# Autodesk Inventor assembly: Finger_L
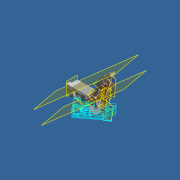
[picture p0: Inventor's stored thumbnail of the model, 180x180]
Saved by Autodesk Inventor 2016 (Build 200138000, 138)
## iProperties
Created: 2015-01-03
Part Number: Finger_L
Document SubType Name: Assembly
Designer: 4ndreas
Author: 4ndreas
## Documents named in this file (17)
- C:\Users\4ndreas\Documents\Inventor\Gripper\3-Finger Gripper\Finger_L.iam
- C:\Users\4ndreas\Documents\Inventor\Gripper\3-Finger Gripper\schnecke.ipt
- C:\Users\4ndreas\Documents\Inventor\Gripper\3-Finger Gripper\DC-Motor_12V_60U-min.ipt
- C:\Users\4ndreas\Documents\Inventor\Gripper\3-Finger Gripper\FingerPartA.ipt
- C:\Users\4ndreas\Documents\Inventor\Gripper\3-Finger Gripper\FingerPartB.ipt
- C:\Users\4ndreas\Documents\Inventor\Gripper\3-Finger Gripper\FingerTipp.ipt
- C:\Users\4ndreas\Documents\Inventor\Gripper\3-Finger Gripper\Hebel_Basis.ipt
- C:\Users\4ndreas\Documents\Inventor\Gripper\3-Finger Gripper\Hebel_Basis 2.ipt
- C:\Users\4ndreas\Documents\Inventor\Gripper\3-Finger Gripper\KippGear_MIR.ipt
- C:\Users\4ndreas\Documents\Inventor\Gripper\3-Finger Gripper\rotMount_MIR.ipt
- C:\Users\4ndreas\Documents\Inventor\Gripper\3-Finger Gripper\deckel_MIR.ipt
- C:\Users\4ndreas\Documents\Inventor\Gripper\3-Finger Gripper\Servo G12DM.ipt
- C:\Users\4ndreas\Documents\Inventor\Gripper\3-Finger Gripper\3_hebenMount_2_dual.ipt
- C:\Users\4ndreas\Documents\Inventor\Gripper\3-Finger Gripper\FingerTip_joint _v2.ipt
- C:\Users\4ndreas\Documents\Inventor\Gripper\3-Finger Gripper\FingerTip_Mount dual.ipt
- C:\Users\4ndreas\Documents\Inventor\Gripper\3-Finger Gripper\Hebel_B dual.ipt
- C:\Users\4ndreas\Documents\Inventor\Gripper\3-Finger Gripper\Hebel_dual.ipt
## Components (18 placed, 16 different names)
1. schnecke:1 — Passend:4, Passend:46, Passend:47
2. DC-Motor_12V_60U-min:1 — Passend:1, Passend:46
3. FingerPartA:1 — Passend:8, Passend:9, Passend:14, Fluchtend:1, Passend:15, Passend:17, Passend:30, Passend:31, Passend:52
4. FingerPartB:1 — Passend:8, Passend:9, Passend:10, Passend:11, Fluchtend:1, Passend:53, Passend:54, Passend:55
5. FingerTipp:1 — Passend:10, Passend:11, Passend:50, Passend:51, Passend:56, Passend:59
6. Hebel_Basis:1 — Passend:14, Passend:16, Passend:23, Passend:63, Passend:64
7. Hebel_Basis 2:1 — Passend:15, Passend:16, Passend:17, Passend:62, Passend:65
8. KippGear_MIR:1 — Passend:25, Passend:26, Passend:33, Passend:34, Passend:35
9. rotMount_MIR:1 — Passend:30, Passend:31, Passend:32, Passend:33, Passend:34, Passend:35, Passend:39, Passend:40, Passend:41, Passend:42, Fluchtend:4, Passend:43, Passend:47, Passend:48, Passend:49, Winkel:1
10. deckel_MIR:1 — Passend:42, Fluchtend:4, Passend:43
11. Servo G12DM:1 — Passend:48, Passend:49, Winkel:1
12. FingerTip_joint _v2:1 — Passend:50, Passend:51, Passend:57, Passend:58
13. 3_hebenMount_2_dual:2 — Passend:52, Passend:53, Passend:61, Passend:66
14. FingerTip_Mount dual:1 — Passend:54, Passend:55, Passend:60, Passend:67
15. Hebel_B dual:1 — Passend:56, Passend:59, Passend:60
16. Hebel_B dual:2 — Passend:57, Passend:58, Passend:61
17. Hebel_dual:1 — Passend:62, Passend:65, Passend:66
18. Hebel_dual:2 — Passend:63, Passend:64, Passend:67
## Relationships (51: Mate 47, Flush 3, Angle 1)
- Passend:1 [Mate]: DC-Motor_12V_60U-min:1
- Passend:4 [Mate]: schnecke:1
- Passend:8 [Mate]: FingerPartA:1 ↔ FingerPartB:1
- Passend:9 [Mate]: FingerPartA:1 ↔ FingerPartB:1
- Passend:10 [Mate]: FingerPartB:1 ↔ FingerTipp:1
- Passend:11 [Mate]: FingerPartB:1 ↔ FingerTipp:1
- Passend:14 [Mate]: FingerPartA:1 ↔ Hebel_Basis:1
- Fluchtend:1 [Flush]: FingerPartA:1 ↔ FingerPartB:1
- Passend:15 [Mate]: FingerPartA:1 ↔ Hebel_Basis 2:1
- Passend:16 [Mate]: Hebel_Basis:1 ↔ Hebel_Basis 2:1
- Passend:17 [Mate]: FingerPartA:1 ↔ Hebel_Basis 2:1
- Passend:23 [Mate]: Hebel_Basis:1
- Fluchtend:2 [Flush] (36.5 mm)
- Passend:25 [Mate]: KippGear_MIR:1
- Passend:26 [Mate]: KippGear_MIR:1
- Passend:29 [Mate]
- Passend:30 [Mate]: FingerPartA:1 ↔ rotMount_MIR:1
- Passend:31 [Mate]: FingerPartA:1 ↔ rotMount_MIR:1
- Passend:32 [Mate]: rotMount_MIR:1
- Passend:33 [Mate]: KippGear_MIR:1 ↔ rotMount_MIR:1
- Passend:34 [Mate]: KippGear_MIR:1 ↔ rotMount_MIR:1
- Passend:35 [Mate]: KippGear_MIR:1 ↔ rotMount_MIR:1
- Passend:39 [Mate]: rotMount_MIR:1
- Passend:40 [Mate]: rotMount_MIR:1
- Passend:41 [Mate]: rotMount_MIR:1
- Passend:42 [Mate]: rotMount_MIR:1 ↔ deckel_MIR:1
- Fluchtend:4 [Flush]: rotMount_MIR:1 ↔ deckel_MIR:1
- Passend:43 [Mate]: rotMount_MIR:1 ↔ deckel_MIR:1
- Passend:46 [Mate] (1 mm): schnecke:1 ↔ DC-Motor_12V_60U-min:1
- Passend:47 [Mate]: schnecke:1 ↔ rotMount_MIR:1
- Passend:48 [Mate]: rotMount_MIR:1 ↔ Servo G12DM:1
- Passend:49 [Mate]: rotMount_MIR:1 ↔ Servo G12DM:1
- Winkel:1 [Angle] (180 deg): rotMount_MIR:1 ↔ Servo G12DM:1
- Passend:50 [Mate]: FingerTipp:1 ↔ FingerTip_joint _v2:1
- Passend:51 [Mate]: FingerTipp:1 ↔ FingerTip_joint _v2:1
- Passend:52 [Mate]: FingerPartA:1 ↔ 3_hebenMount_2_dual:2
- Passend:53 [Mate]: FingerPartB:1 ↔ 3_hebenMount_2_dual:2
- Passend:54 [Mate]: FingerPartB:1 ↔ FingerTip_Mount dual:1
- Passend:55 [Mate]: FingerPartB:1 ↔ FingerTip_Mount dual:1
- Passend:56 [Mate]: FingerTipp:1 ↔ Hebel_B dual:1
- Passend:57 [Mate]: FingerTip_joint _v2:1 ↔ Hebel_B dual:2
- Passend:58 [Mate]: FingerTip_joint _v2:1 ↔ Hebel_B dual:2
- Passend:59 [Mate]: FingerTipp:1 ↔ Hebel_B dual:1
- Passend:60 [Mate]: FingerTip_Mount dual:1 ↔ Hebel_B dual:1
- Passend:61 [Mate]: 3_hebenMount_2_dual:2 ↔ Hebel_B dual:2
- Passend:62 [Mate]: Hebel_Basis 2:1 ↔ Hebel_dual:1
- Passend:63 [Mate]: Hebel_Basis:1 ↔ Hebel_dual:2
- Passend:64 [Mate]: Hebel_Basis:1 ↔ Hebel_dual:2
- Passend:65 [Mate]: Hebel_Basis 2:1 ↔ Hebel_dual:1
- Passend:66 [Mate]: 3_hebenMount_2_dual:2 ↔ Hebel_dual:1
- Passend:67 [Mate]: FingerTip_Mount dual:1 ↔ Hebel_dual:2
